# Autodesk Inventor assembly: obj5
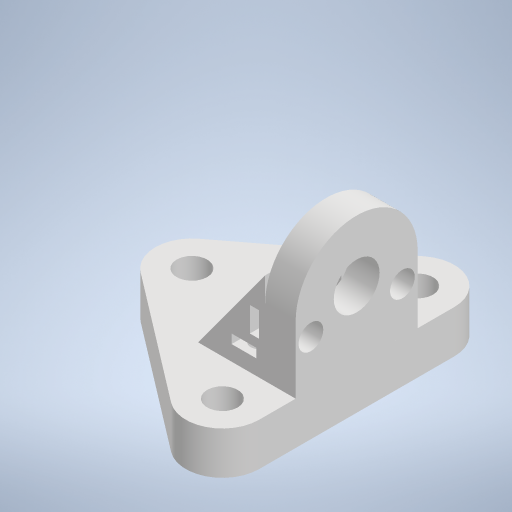
[picture p0: Inventor's stored thumbnail of the model, 512x512]
Saved by Autodesk Inventor 2023.2 (Build 272271030, 271C)
## iProperties
Created: 2023-02-25
Part Number: obj5
Document SubType Name: Assembly
Designer: Cris Pat
Author: Cris Pat
## Documents named in this file (4)
- C:\Users\Cris Pat\Desktop\U\Semestre 9\disenio e innovacion\CAD\obj5.iam
- C:\Users\Cris Pat\Desktop\U\Semestre 9\disenio e innovacion\CAD\arco_obj4.ipt
- C:\Users\Cris Pat\Desktop\U\Semestre 9\disenio e innovacion\CAD\base_obj4.ipt
- C:\Users\Cris Pat\Desktop\U\Semestre 9\disenio e innovacion\CAD\ligamento_obj4.ipt
## Components (4 placed, 3 different names)
1. arco_obj4:1 — Rigid:1, Rigid:2
2. base_obj4:1 — Rotational:1
3. ligamento_obj4:1 — Rigid:1
4. ligamento_obj4:2 — Rigid:2, Rotational:1
## Relationships (3: WeldJoint 2, RevoluteJoint 1)
- Rigid:1 [WeldJoint]: arco_obj4:1 ↔ ligamento_obj4:1
- Rigid:2 [WeldJoint]: arco_obj4:1 ↔ ligamento_obj4:2
- Rotational:1 [RevoluteJoint]: base_obj4:1 ↔ ligamento_obj4:2
